# Autodesk Inventor assembly: frame
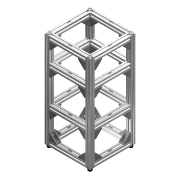
[picture p0: Inventor's stored thumbnail of the model, 180x180]
Saved by Autodesk Inventor 2017 (Build 210142000, 142)
## iProperties
Created: 2016-07-21
Part Number: frame
Document SubType Name: Assembly
Designer: Jonathan
Author: Jonathan
## Documents named in this file (6)
- C:\Users\sawaiz\oneDrive\projects\muonTelescope\frame\frame.iam
- C:\Users\sawaiz\oneDrive\projects\muonTelescope\frame\shapes\15x15.iam
- C:\Users\sawaiz\oneDrive\projects\muonTelescope\frame\extrusions\40 cm extrusion.ipt
- C:\Users\sawaiz\oneDrive\projects\muonTelescope\frame\feet\m5x25.ipt
- C:\Users\sawaiz\oneDrive\projects\muonTelescope\frame\feet\roundBumper.ipt
- C:\Users\sawaiz\oneDrive\projects\muonTelescope\frameSpecifications.xlsx
## Components (16 placed, 4 different names)
1. 15x15:1 [sub-assembly] — Mate:1, Mate:2, Flush:1, Mate:3, Mate:4, Flush:2, Mate:5, Mate:6, Flush:3, Mate:7, Mate:8, Flush:4, Flush:6
2. 40 cm extrusion:1 — Mate:3, Mate:4, Flush:2, Symmetry:2, Symmetry:3, Mate:23, Mate:27
3. 40 cm extrusion:2 — Mate:1, Mate:2, Flush:1, Symmetry:3, Mate:26
4. 40 cm extrusion:3 — Mate:7, Mate:8, Flush:4, Mate:9, Mate:10, Flush:5, Mate:11, Mate:12, Mate:13, Mate:14, Symmetry:1, Symmetry:2, Mate:24
5. 40 cm extrusion:4 — Mate:5, Mate:6, Flush:3, Symmetry:1, Mate:25
6. 15x15:2 [sub-assembly] — Mate:9, Mate:10, Flush:5
7. 15x15:3 [sub-assembly] — Mate:12, Mate:13, Flush:7
8. 15x15:4 [sub-assembly] — Mate:11, Mate:14, Flush:6, Flush:7
9. m5x25:1 — Mate:24
10. roundBumper:1 — Flush:9, Flush:10
11. m5x25:2 — Mate:23
12. roundBumper:2 — Flush:10, Mate:27
13. m5x25:3 — Mate:26
14. roundBumper:3 — Flush:8
15. m5x25:4 — Mate:25
16. roundBumper:4 — Flush:8, Flush:9
## Relationships (40: Mate 27, Flush 10, Symmetry 3)
- Mate:1: 15x15:1 ↔ 40 cm extrusion:2
- Mate:2: 15x15:1 ↔ 40 cm extrusion:2
- Flush:1: 15x15:1 ↔ 40 cm extrusion:2
- Mate:3: 15x15:1 ↔ 40 cm extrusion:1
- Mate:4: 15x15:1 ↔ 40 cm extrusion:1
- Flush:2: 15x15:1 ↔ 40 cm extrusion:1
- Mate:5: 15x15:1 ↔ 40 cm extrusion:4
- Mate:6: 15x15:1 ↔ 40 cm extrusion:4
- Flush:3: 15x15:1 ↔ 40 cm extrusion:4
- Mate:7: 15x15:1 ↔ 40 cm extrusion:3
- Mate:8: 15x15:1 ↔ 40 cm extrusion:3
- Flush:4: 15x15:1 ↔ 40 cm extrusion:3
- Mate:9: 40 cm extrusion:3 ↔ 15x15:2
- Mate:10: 40 cm extrusion:3 ↔ 15x15:2
- Flush:5: 40 cm extrusion:3 ↔ 15x15:2
- Mate:11: 40 cm extrusion:3 ↔ 15x15:4
- Mate:12: 40 cm extrusion:3 ↔ 15x15:3
- Mate:13: 40 cm extrusion:3 ↔ 15x15:3
- Mate:14: 40 cm extrusion:3 ↔ 15x15:4
- Flush:6 (100 mm): 15x15:1 ↔ 15x15:4
- Flush:7 (-150 mm): 15x15:3 ↔ 15x15:4
- Symmetry:1: 40 cm extrusion:3 ↔ 40 cm extrusion:4
- Symmetry:2: 40 cm extrusion:1 ↔ 40 cm extrusion:3
- Symmetry:3: 40 cm extrusion:1 ↔ 40 cm extrusion:2
- [Mate]: m5x25:1 ↔ roundBumper:1
- [Mate]: m5x25:1 ↔ roundBumper:1
- [Mate]: m5x25:2 ↔ roundBumper:2
- [Mate]: m5x25:2 ↔ roundBumper:2
- [Mate]: m5x25:3 ↔ roundBumper:3
- [Mate]: m5x25:3 ↔ roundBumper:3
- [Mate]: m5x25:4 ↔ roundBumper:4
- [Mate]: m5x25:4 ↔ roundBumper:4
- Mate:23: 40 cm extrusion:1 ↔ m5x25:2
- Mate:24: 40 cm extrusion:3 ↔ m5x25:1
- Mate:25: 40 cm extrusion:4 ↔ m5x25:4
- Mate:26: 40 cm extrusion:2 ↔ m5x25:3
- Flush:8: roundBumper:3 ↔ roundBumper:4
- Flush:9: roundBumper:1 ↔ roundBumper:4
- Flush:10: roundBumper:1 ↔ roundBumper:2
- Mate:27: 40 cm extrusion:1 ↔ roundBumper:2
## Named parameters: height = 400 mm, width = 150 mm, topSeparation = 100 mm, botSeparation = 150 mm, panelChamfer = 75 mm, suppourtPanelThickness = 2.38125 mm, d23_d39 = 0 mm, d24_d40 = 0 mm, d25_d39 = 0 mm, d26_d40 = 0 mm, d27_d39 = 0 mm, d28_d40 = 0 mm
